# Autodesk Inventor assembly: R-T v4
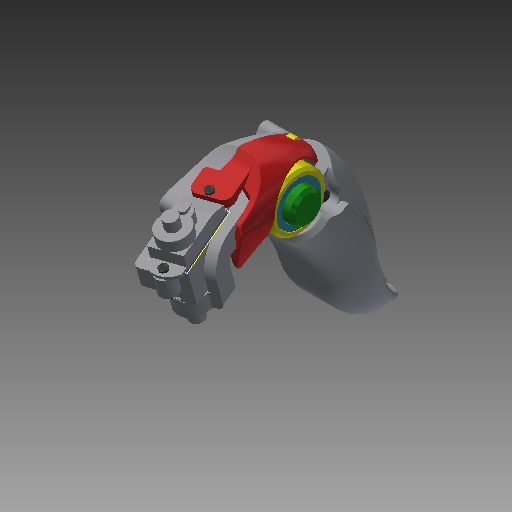
[picture p0: Inventor's stored thumbnail of the model, 512x512]
Saved by Autodesk Inventor 2018 (Build 220112000, 112)
## iProperties
Created: 2017-09-22
Part Number: R-T v4
Material: 一般
Document SubType Name: Assembly
Designer: sktom
Author: sktom
## Documents named in this file (9)
- D:\cloudstrage\NextCloud\Cad_mechanical\HACKberry_SizeM\3Dmodel\R\M-R-H\M-R-T\M-R-T.iam
- D:\cloudstrage\NextCloud\Cad_mechanical\HACKberry_SizeM\3Dmodel\R\M-R-H\M-R-T\M-R-T-03.ipt
- D:\cloudstrage\NextCloud\Cad_mechanical\HACKberry_SizeM\3Dmodel\R\M-R-H\M-R-T\M-R-T-02.ipt
- D:\cloudstrage\NextCloud\Cad_mechanical\HACKberry_SizeM\3Dmodel\R\M-R-H\M-R-T\M-R-T-01.ipt
- D:\cloudstrage\NextCloud\Cad_mechanical\HACKberry_SizeM\3Dmodel\R\M-R-H\M-R-T\M-R-T-04.ipt
- D:\cloudstrage\NextCloud\Cad_mechanical\HACKberry_SizeM\3Dmodel\R\M-R-H\M-R-T\M-R-T-05.ipt
- D:\cloudstrage\NextCloud\Cad_mechanical\HACKberry_SizeM\3Dmodel\R\M-R-H\M-R-T\M-R-T-06.ipt
- D:\cloudstrage\NextCloud\Cad_mechanical\HACKberry_SizeM\3Dmodel\R\M-R-H\M-R-T\Servo_HK282A.ipt
- D:\cloudstrage\NextCloud\Cad_mechanical\HACKberry_SizeM\3Dmodel\R\M-R-H\M-R-T\M1.7_L8.ipt
## Components (12 placed, 8 different names)
1. R-T-03 v1:1 — 回転:3, リジッド:1
2. R-T-01 v1:1 — 角度:1, 挿入:5
3. R-T-02 v1:1 — 回転:3, 角度:1
4. R-T-04 v1:1 — リジッド:1
5. R-T-05 v1:1 — 円柱状:2, 挿入:3, 挿入:4
6. R-T-06 v1:1 — 円柱状:2, 挿入:2
7. Servo_HK282A:1 — 挿入:1
8. M1.7_L8:1 — 挿入:1
9. M1.7_L8:2 — 挿入:2
10. M1.7_L8:3 — 挿入:3
11. M1.7_L8:4 — 挿入:4
12. M1.7_L8:5 — 挿入:5
## Relationships (9: Insert 5, RevoluteJoint 1, Angle 1, WeldJoint 1, CylindricalJoint 1)
- 回転:3 [RevoluteJoint] (-0.3 mm): R-T-03 v1:1 ↔ R-T-02 v1:1
- 角度:1 [Angle] (180 deg): R-T-01 v1:1 ↔ R-T-02 v1:1
- リジッド:1 [WeldJoint] (3 mm): R-T-03 v1:1 ↔ R-T-04 v1:1
- 円柱状:2 [CylindricalJoint]: R-T-05 v1:1 ↔ R-T-06 v1:1
- 挿入:1 [Insert]: Servo_HK282A:1 ↔ M1.7_L8:1
- 挿入:2 [Insert]: R-T-06 v1:1 ↔ M1.7_L8:2
- 挿入:3 [Insert]: R-T-05 v1:1 ↔ M1.7_L8:3
- 挿入:4 [Insert]: R-T-05 v1:1 ↔ M1.7_L8:4
- 挿入:5 [Insert]: R-T-01 v1:1 ↔ M1.7_L8:5
